# Autodesk Inventor assembly: Assembly new
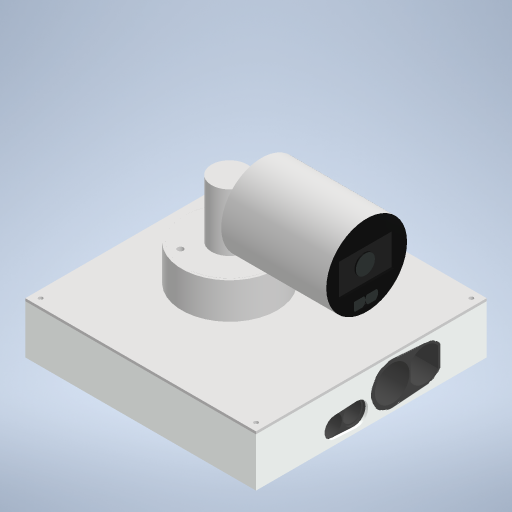
[picture p0: Inventor's stored thumbnail of the model, 512x512]
Saved by Autodesk Inventor 2024.1 (Build 281209000, 209)
## iProperties
Created: 2026-03-19
Part Number: Assembly new
Document SubType Name: Assembly
Designer: User
Author: User
## Documents named in this file (7)
- C:\Users\User\Downloads\capstone\Assembly new.iam
- C:\Users\User\Downloads\capstone\base plate new.ipt
- C:\Users\User\Downloads\capstone\top plate - new.ipt
- C:\Users\User\Downloads\capstone\Big LRF Real.ipt
- C:\Users\User\Downloads\capstone\Small LRF Real.ipt
- C:\Users\User\Downloads\capstone\camera real.ipt
- C:\Users\User\Downloads\capstone\USB hub.ipt
## Components (6 placed, 6 different names)
1. base plate new:1 — Flush:2, Mate:1, Mate:2, Insert:1, Mate:3, Flush:3, Flush:4, Mate:4, Mate:5
2. top plate - new:1 — Mate:3, Flush:3, Flush:4, Insert:2, Insert:3
3. Big LRF Real:1 — Flush:2
4. Small LRF Real:1 — Mate:1, Mate:2, Insert:1
5. camera real:1 — Insert:2, Insert:3
6. USB hub:1 — Mate:4, Mate:5
## Relationships (11: Mate 5, Flush 3, Insert 3)
- Flush:2: base plate new:1 ↔ Big LRF Real:1
- Mate:1: base plate new:1 ↔ Small LRF Real:1
- Mate:2: base plate new:1 ↔ Small LRF Real:1
- Insert:1: base plate new:1 ↔ Small LRF Real:1
- Mate:3: base plate new:1 ↔ top plate - new:1
- Flush:3: base plate new:1 ↔ top plate - new:1
- Flush:4: base plate new:1 ↔ top plate - new:1
- Insert:2: top plate - new:1 ↔ camera real:1
- Insert:3: top plate - new:1 ↔ camera real:1
- Mate:4: base plate new:1 ↔ USB hub:1
- Mate:5: base plate new:1 ↔ USB hub:1
